# Autodesk Inventor assembly: actuator_second
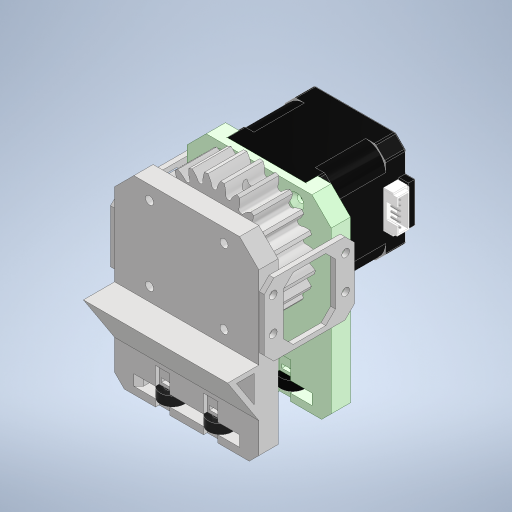
[picture p0: Inventor's stored thumbnail of the model, 512x512]
Saved by Autodesk Inventor 2023.1 (Build 271208000, 208)
## iProperties
Created: 2025-12-13
Part Number: actuator_second
Document SubType Name: Assembly
Designer: DELL
Author: DELL
## Documents named in this file (9)
- C:\Users\DELL\reposGitHub\VSOSH25-26\models\actuator\actuator_second.iam
- C:\Users\DELL\reposGitHub\VSOSH25-26\models\import\Schrittmotor-42SHDC3025-24B.ipt
- C:\Users\DELL\reposGitHub\VSOSH25-26\models\actuator\звезда_шестрерни.ipt
- C:\Users\DELL\reposGitHub\VSOSH25-26\models\actuator\муфта.ipt
- C:\Users\DELL\reposGitHub\VSOSH25-26\models\actuator\шестреня_12.12.ipt
- C:\Users\DELL\reposGitHub\VSOSH25-26\models\actuator\каретка.ipt
- C:\Users\DELL\reposGitHub\VSOSH25-26\models\actuator\колесико.ipt
- C:\Users\DELL\reposGitHub\VSOSH25-26\models\actuator\стена_простая.ipt
- C:\Users\DELL\reposGitHub\VSOSH25-26\models\actuator\каретка_м3_без_м.ipt
## Components (12 placed, 8 different names)
1. Schrittmotor-42SHDC3025-24B:1 — Заподлицо:1, Совмещение:1, Совмещение:2, Совмещение:4, Заподлицо:3
2. звезда_шестрерни:1 — Совмещение:5, Совмещение:6, Совмещение:7, Совмещение:8, Заподлицо:2
3. муфта:1 — Совмещение:4, Совмещение:5, Совмещение:6, Совмещение:9
4. шестреня_12.12:1 — Совмещение:7, Совмещение:8, Заподлицо:2
5. каретка:1 — Заподлицо:3, Совмещение:9, Совмещение:30, Совмещение:31, Совмещение:32, Совмещение:37, Совмещение:41, Совмещение:43, Совмещение:52, Совмещение:53
6. колесико:2 — Совмещение:43, Совмещение:53
7. стена_простая:1 — Совмещение:30, Совмещение:31, Совмещение:32, Совмещение:54, Совмещение:55, Совмещение:56
8. стена_простая:2 — Совмещение:37
9. колесико:6 — Совмещение:41, Совмещение:52
10. каретка_м3_без_м:1 — Совмещение:54, Совмещение:55, Совмещение:56, Совмещение:57, Совмещение:58, Совмещение:59, Совмещение:60
11. колесико:7 — Совмещение:59, Совмещение:60
12. колесико:8 — Совмещение:57, Совмещение:58
## Relationships (26: Mate 23, Flush 3)
- Заподлицо:1 [Flush]: Schrittmotor-42SHDC3025-24B:1
- Совмещение:1 [Mate]: Schrittmotor-42SHDC3025-24B:1
- Совмещение:2 [Mate]: Schrittmotor-42SHDC3025-24B:1
- Совмещение:4 [Mate]: Schrittmotor-42SHDC3025-24B:1 ↔ муфта:1
- Совмещение:5 [Mate]: звезда_шестрерни:1 ↔ муфта:1
- Совмещение:6 [Mate]: звезда_шестрерни:1 ↔ муфта:1
- Совмещение:7 [Mate]: звезда_шестрерни:1 ↔ шестреня_12.12:1
- Совмещение:8 [Mate]: звезда_шестрерни:1 ↔ шестреня_12.12:1
- Заподлицо:2 [Flush]: звезда_шестрерни:1 ↔ шестреня_12.12:1
- Заподлицо:3 [Flush]: Schrittmotor-42SHDC3025-24B:1 ↔ каретка:1
- Совмещение:9 [Mate] (0.5 mm): муфта:1 ↔ каретка:1
- Совмещение:30 [Mate]: каретка:1 ↔ стена_простая:1
- Совмещение:31 [Mate]: каретка:1 ↔ стена_простая:1
- Совмещение:32 [Mate]: каретка:1 ↔ стена_простая:1
- Совмещение:37 [Mate]: каретка:1 ↔ стена_простая:2
- Совмещение:41 [Mate]: каретка:1 ↔ колесико:6
- Совмещение:43 [Mate]: каретка:1 ↔ колесико:2
- Совмещение:52 [Mate]: каретка:1 ↔ колесико:6
- Совмещение:53 [Mate]: каретка:1 ↔ колесико:2
- Совмещение:54 [Mate]: стена_простая:1 ↔ каретка_м3_без_м:1
- Совмещение:55 [Mate]: стена_простая:1 ↔ каретка_м3_без_м:1
- Совмещение:56 [Mate]: стена_простая:1 ↔ каретка_м3_без_м:1
- Совмещение:57 [Mate]: каретка_м3_без_м:1 ↔ колесико:8
- Совмещение:58 [Mate]: каретка_м3_без_м:1 ↔ колесико:8
- Совмещение:59 [Mate]: каретка_м3_без_м:1 ↔ колесико:7
- Совмещение:60 [Mate]: каретка_м3_без_м:1 ↔ колесико:7
